# Autodesk Inventor assembly: tower
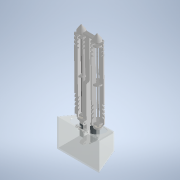
[picture p0: Inventor's stored thumbnail of the model, 180x180]
Saved by Autodesk Inventor 2020.1 (Build 241239000, 239)
## iProperties
Created: 2022-03-22
Part Number: tower
Document SubType Name: Assembly
Designer: User
Author: User
## Documents named in this file (5)
- D:\GitHub\TANK\3D-turret\tower 2.iam
- D:\GitHub\TANK\3D-turret\корпус башни.ipt
- D:\GitHub\TANK\3D-turret\ось крепление пушки.ipt
- D:\GitHub\TANK\3D-turret\MG996R.ipt
- D:\GitHub\TANK\3D-turret\full guns 4.iam
## Components (4 placed, 4 different names)
1. корпус башни:1 — С поворотом:1
2. ось крепление пушки:1 — С поворотом:1, Совмещение:1
3. MG996R:1
4. full guns 4:1 [sub-assembly] — Совмещение:1
## Relationships (2: RevoluteJoint 1, Mate 1)
- С поворотом:1 [RevoluteJoint]: корпус башни:1 ↔ ось крепление пушки:1
- Совмещение:1 [Mate]: ось крепление пушки:1 ↔ full guns 4:1
